# Autodesk Inventor assembly: setup
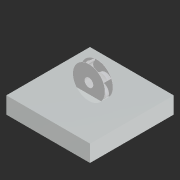
[picture p0: Inventor's stored thumbnail of the model, 180x180]
Saved by Autodesk Inventor 2020.3 (Build 243373010, 373A)
## iProperties
Created: 2020-12-30
Part Number: setup
Document SubType Name: Assembly
Designer: Melvin Strobl
Author: Melvin Strobl
## Documents named in this file (3)
- X:\waterturbine\setup.iam
- X:\waterturbine\watertubine_b.ipt
- X:\waterturbine\tunnel.ipt
## Components (2 placed, 2 different names)
1. watertubine_b:1 — Mate:1, Mate:3
2. tunnel:1 — Mate:2, Flush:1
## Relationships (4: Mate 3, Flush 1)
- Mate:1: watertubine_b:1
- Mate:2 (-150 mm): tunnel:1
- Mate:3 (10 mm): watertubine_b:1
- Flush:1 (-200 mm): tunnel:1
